# Autodesk Inventor assembly: Body Cover Assembly
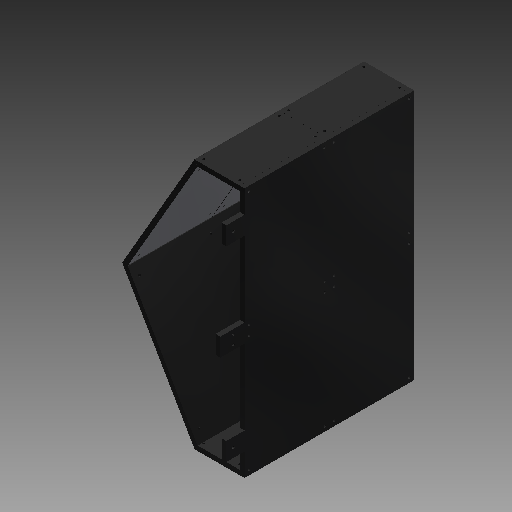
[picture p0: Inventor's stored thumbnail of the model, 512x512]
Saved by Autodesk Inventor 2017 (Build 210142000, 142)
## iProperties
Created: 2018-10-18
Part Number: Body Cover Assembly
Document SubType Name: Assembly
Designer: Dell
Author: Dell
## Documents named in this file (5)
- C:\Users\Dell\Documents\GitHub\tr2\Body\Body Cover Assembly.iam
- C:\Users\Dell\Documents\GitHub\tr2\Body\BO07.ipt
- C:\Users\Dell\Documents\GitHub\tr2\Body\BO08.ipt
- C:\Users\Dell\Documents\GitHub\tr2\Body\BO09.ipt
- C:\Users\Dell\Documents\GitHub\tr2\Body\BO10.ipt
## Components (12 placed, 4 different names)
1. BO07:1
2. BO08:1
3. BO09:1
4. BO09:2
5. BO08:2
6. BO08:3
7. BO08:4
8. BO07:2
9. BO07:3
10. BO07:4
11. BO10:1
12. BO10:2
## Relationships (18: Mate 15, Flush 3)
- [Mate]: BO09:1 ↔ BO09:2
- [Mate]: BO08:1 ↔ BO09:1
- [Mate]: BO08:1 ↔ BO09:1
- [Mate]: BO07:1 ↔ BO08:1
- [Mate]: BO08:1 ↔ BO08:2
- [Mate]: BO09:1 ↔ BO08:2
- [Mate]: BO09:2 ↔ BO08:3
- [Mate]: BO08:3 ↔ BO08:4
- [Mate]: BO08:3 ↔ BO08:4
- [Mate]: BO07:1 ↔ BO07:2
- [Mate]: BO07:1 ↔ BO07:3
- [Mate]: BO08:2 ↔ BO07:3
- [Mate]: BO07:3 ↔ BO07:4
- [Flush]: BO07:3 ↔ BO07:4
- [Mate]: BO09:2 ↔ BO10:1
- [Flush]: BO09:1 ↔ BO10:1
- [Mate]: BO09:2 ↔ BO10:2
- [Flush]: BO09:2 ↔ BO10:2
